# Autodesk Inventor assembly: mesoSPIM(v4-5)DetectionArmUpgrade2023
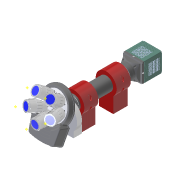
[picture p0: Inventor's stored thumbnail of the model, 180x180]
Saved by Autodesk Inventor 2021 (Build 250183000, 183)
## iProperties
Created: 2023-03-17
Part Number: mesoSPIM(v4-5)DetectionArmUpgrade2023
Document SubType Name: Assembly
Designer: nvladi
Author: nvladi
## Documents named in this file (12)
- C:\Users\Public\GitHub-public\benchtop-hardware\v4-5-upgrade-2023\CAD-AutodeskInventor2021\mesoSPIM(v4-5)DetectionArmUpgrade2023.iam
- C:\Users\Public\GitHub-public\benchtop-hardware\v4-5-upgrade-2023\CAD-AutodeskInventor2021\Mitutoyo-5pos-726.iam
- C:\Users\Public\GitHub-public\benchtop-hardware\v4-5-upgrade-2023\custom-parts\MotorizedRevolver\MotorizedRevolver-SM2-adapter.ipt
- C:\Users\Public\GitHub-public\benchtop-hardware\Benchtop\CAD-model-Inventor2021\library\Thorlabs\lens_tubes\SM2L10.ipt
- C:\Users\Public\GitHub-public\benchtop-hardware\Benchtop\CAD-model-Inventor2021\library\Thorlabs\accessoires\TMA4.ipt
- C:\Users\Public\GitHub-public\benchtop-hardware\Benchtop\CAD-model-Inventor2021\library\ZWO-EWF(filter_wheel)\ZWO-EFW-Mini.ipt
- C:\Users\Public\GitHub-public\benchtop-hardware\Benchtop\CAD-model-Inventor2021\library\Thorlabs\lens_tubes\SM2E60.ipt
- C:\Users\Public\GitHub-public\benchtop-hardware\Benchtop\CAD-model-Inventor2021\library\Thorlabs\accessoires\SM2T2.ipt
- C:\Users\Public\GitHub-public\benchtop-hardware\Benchtop\CAD-model-Inventor2021\library\Thorlabs\lens_tubes\SM2M20.ipt
- C:\Users\Public\GitHub-public\benchtop-hardware\Benchtop\CAD-model-Inventor2021\library\Thorlabs\f-mounts\SM2NFM2.ipt
- C:\Users\Public\GitHub-public\benchtop-hardware\v4-5-upgrade-2023\custom-parts\RailMounting\ThorlabsSM2L30-XT66P2M_H94mm(axis2base).ipt
- C:\Users\Public\GitHub-public\benchtop-hardware\Benchtop\CAD-model-Inventor2021\library\Photometrics\Iris15_Volume_Correct.ipt
## Components (13 placed, 11 different names)
1. Mitutoyo-5pos-726:1 [sub-assembly] — Insert:1
2. MotorizedRevolver-SM2-adapter:1 — Insert:1, Insert:2
3. SM2L10:1 — Insert:2, Insert:3
4. TMA4:1 — Insert:3, Insert:4
5. TMA4:2 — Insert:5, Insert:6
6. ZWO-EFW-Mini:1 — Insert:4, Insert:5, Angle:1
7. SM2E60:1 — Insert:7, Insert:8, Insert:10, Insert:11
8. SM2T2:1 — Insert:6, Insert:7
9. SM2M20:1 — Insert:8, Insert:9
10. SM2NFM2:1 — Insert:9, Insert:12
11. ThorlabsSM2L30-XT66P2M_H94mm(axis2base):1 — Insert:10
12. ThorlabsSM2L30-XT66P2M_H94mm(axis2base):2 — Insert:11
13. Iris15_Volume_Correct:1 — Insert:12
## Relationships (13: Insert 12, Angle 1)
- Insert:1 (2 mm): Mitutoyo-5pos-726:1 ↔ MotorizedRevolver-SM2-adapter:1
- Insert:2: MotorizedRevolver-SM2-adapter:1 ↔ SM2L10:1
- Insert:3: SM2L10:1 ↔ TMA4:1
- Insert:4: TMA4:1 ↔ ZWO-EFW-Mini:1
- Insert:5: TMA4:2 ↔ ZWO-EFW-Mini:1
- Angle:1 (0 deg): ZWO-EFW-Mini:1
- Insert:6: TMA4:2 ↔ SM2T2:1
- Insert:7: SM2E60:1 ↔ SM2T2:1
- Insert:8 (1 mm): SM2E60:1 ↔ SM2M20:1
- Insert:9: SM2M20:1 ↔ SM2NFM2:1
- Insert:10 (5 mm): SM2E60:1 ↔ ThorlabsSM2L30-XT66P2M_H94mm(axis2base):1
- Insert:11 (-15 mm): SM2E60:1 ↔ ThorlabsSM2L30-XT66P2M_H94mm(axis2base):2
- Insert:12: SM2NFM2:1 ↔ Iris15_Volume_Correct:1
